# Autodesk Inventor assembly: MainDriveTestRig
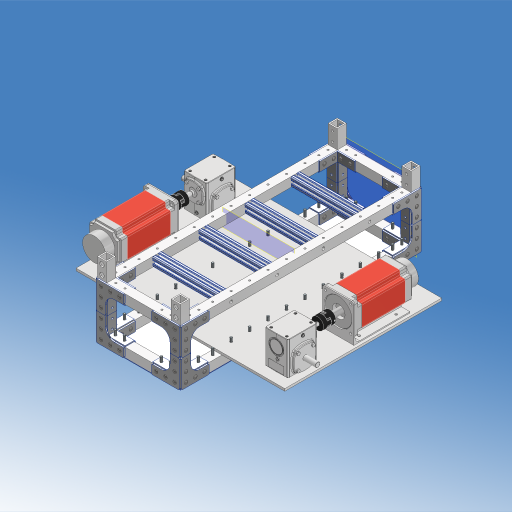
[picture p0: Inventor's stored thumbnail of the model, 512x512]
Saved by Autodesk Inventor 2024 (Build 280153000, 153)
## iProperties
Created: 2024-02-14
Part Number: MainDriveTestRig
Document SubType Name: Assembly
Designer: seene
Author: seene
## Documents named in this file (10)
- C:\Users\seene\OneDrive\SBRT\Robocup Rescue\Drive\TestRigs\MainDriveTestrig\MainDriveTestRig.iam
- C:\Users\seene\OneDrive\SBRT\Robocup Rescue\Chassis\Frame\Centerpiece\Centerpiece_Frame.iam
- Centerpiece_Frame.iam
- C:\Users\seene\OneDrive\SBRT\Robocup Rescue\Drive\v1\QCI-34HC-3_v2.ipt
- C:\Users\seene\OneDrive\SBRT\Robocup Rescue\Drive\v1\5887K171_Right-Angle Speed Reducer.ipt
- C:\Users\seene\OneDrive\SBRT\Robocup Rescue\Drive\v1\9939T12_Durometer 64D Spider for 1-5 16 OD Set Screw Vibrate-Damping Precision Flexible Shaft Coupling.ipt
- C:\Users\seene\OneDrive\SBRT\Robocup Rescue\Drive\v1\9939T102_Vibrate-Damping Precision Flexible Shaft Coupling.ipt
- C:\Users\seene\OneDrive\SBRT\Robocup Rescue\Drive\v1\9939T104_Vibrate-Damping Precision Flexible Shaft Coupling.ipt
- C:\Users\seene\OneDrive\SBRT\Robocup Rescue\Drive\TestRigs\MainDriveTestrig\MotorAttachementPlate.ipt
- C:\Users\seene\OneDrive\SBRT\Robocup Rescue\Drive\TestRigs\MainDriveTestrig\MotorStandoff.ipt
## Components (14 placed, 8 different names)
1. Centerpiece_Frame:1 [sub-assembly] — Mate:22, Mate:23, Mate:24
2. QCI-34HC-3_v2:2 — Rigid:1, Mate:21, Angle:1, Symmetry:2, Flush:30, Mate:30, Mate:31
3. 5887K171_Right-Angle Speed Reducer:1 — Mate:6, Mate:7, Flush:7, Mate:26, Flush:8
4. 9939T102_Vibrate-Damping Precision Flexible Shaft Coupling:1 — Mate:1, Mate:2, Mate:3, Mate:4, Mate:6, Mate:7
5. 9939T104_Vibrate-Damping Precision Flexible Shaft Coupling:1 — Mate:1, Mate:2, Mate:5, Rigid:1
6. 9939T12_Durometer 64D Spider for 1-5 16 OD Set Screw Vibrate-Damping Precision Flexible Shaft Coupling:2 — Mate:3, Mate:4, Mate:5
7. QCI-34HC-3_v2:3 — Mate:19, Mate:20, Symmetry:1, Mate:25, Flush:29, Mate:29
8. 5887K171_Right-Angle Speed Reducer:3 — Flush:3, Flush:6, Mate:27
9. 9939T102_Vibrate-Damping Precision Flexible Shaft Coupling:3
10. 9939T104_Vibrate-Damping Precision Flexible Shaft Coupling:3
11. 9939T12_Durometer 64D Spider for 1-5 16 OD Set Screw Vibrate-Damping Precision Flexible Shaft Coupling:3
12. MotorAttachementPlate:1 — Mate:22, Mate:23, Mate:24, Mate:25, Flush:6, Flush:7, Mate:26, Mate:27, Flush:8
13. MotorStandoff:1 — Flush:29, Mate:29
14. MotorStandoff:2 — Flush:30, Mate:30, Mate:31
## Relationships (39: Mate 26, Flush 8, WeldJoint 2, Symmetry 2, Angle 1)
- Mate:1: 9939T102_Vibrate-Damping Precision Flexible Shaft Coupling:1 ↔ 9939T104_Vibrate-Damping Precision Flexible Shaft Coupling:1
- Mate:2: 9939T102_Vibrate-Damping Precision Flexible Shaft Coupling:1 ↔ 9939T104_Vibrate-Damping Precision Flexible Shaft Coupling:1
- Mate:3: 9939T102_Vibrate-Damping Precision Flexible Shaft Coupling:1 ↔ 9939T12_Durometer 64D Spider for 1-5 16 OD Set Screw Vibrate-Damping Precision Flexible Shaft Coupling:2
- Mate:4: 9939T102_Vibrate-Damping Precision Flexible Shaft Coupling:1 ↔ 9939T12_Durometer 64D Spider for 1-5 16 OD Set Screw Vibrate-Damping Precision Flexible Shaft Coupling:2
- Mate:5: 9939T104_Vibrate-Damping Precision Flexible Shaft Coupling:1 ↔ 9939T12_Durometer 64D Spider for 1-5 16 OD Set Screw Vibrate-Damping Precision Flexible Shaft Coupling:2
- Rigid:1 [WeldJoint]: QCI-34HC-3_v2:2 ↔ 9939T104_Vibrate-Damping Precision Flexible Shaft Coupling:1
- Mate:6: 5887K171_Right-Angle Speed Reducer:1 ↔ 9939T102_Vibrate-Damping Precision Flexible Shaft Coupling:1
- Mate:7: 5887K171_Right-Angle Speed Reducer:1 ↔ 9939T102_Vibrate-Damping Precision Flexible Shaft Coupling:1
- [Mate]: 9939T102_Vibrate-Damping Precision Flexible Shaft Coupling:3 ↔ 9939T104_Vibrate-Damping Precision Flexible Shaft Coupling:3
- [Mate]: 9939T102_Vibrate-Damping Precision Flexible Shaft Coupling:3 ↔ 9939T104_Vibrate-Damping Precision Flexible Shaft Coupling:3
- [Mate]: 9939T102_Vibrate-Damping Precision Flexible Shaft Coupling:3 ↔ 9939T12_Durometer 64D Spider for 1-5 16 OD Set Screw Vibrate-Damping Precision Flexible Shaft Coupling:3
- [Mate]: 9939T102_Vibrate-Damping Precision Flexible Shaft Coupling:3 ↔ 9939T12_Durometer 64D Spider for 1-5 16 OD Set Screw Vibrate-Damping Precision Flexible Shaft Coupling:3
- [Mate]: 9939T104_Vibrate-Damping Precision Flexible Shaft Coupling:3 ↔ 9939T12_Durometer 64D Spider for 1-5 16 OD Set Screw Vibrate-Damping Precision Flexible Shaft Coupling:3
- [WeldJoint]: QCI-34HC-3_v2:3 ↔ 9939T104_Vibrate-Damping Precision Flexible Shaft Coupling:3
- [Mate]: 5887K171_Right-Angle Speed Reducer:3 ↔ 9939T102_Vibrate-Damping Precision Flexible Shaft Coupling:3
- [Mate]: 5887K171_Right-Angle Speed Reducer:3 ↔ 9939T102_Vibrate-Damping Precision Flexible Shaft Coupling:3
- Mate:19: QCI-34HC-3_v2:3
- Mate:20: QCI-34HC-3_v2:3
- Symmetry:1: QCI-34HC-3_v2:3
- Flush:3 (-33.274 mm): 5887K171_Right-Angle Speed Reducer:3
- Flush:4
- Mate:21: QCI-34HC-3_v2:2
- Angle:1 (0 deg): QCI-34HC-3_v2:2
- Symmetry:2: QCI-34HC-3_v2:2
- Flush:5
- Mate:22: Centerpiece_Frame:1 ↔ MotorAttachementPlate:1
- Mate:23: Centerpiece_Frame:1 ↔ MotorAttachementPlate:1
- Mate:24: Centerpiece_Frame:1 ↔ MotorAttachementPlate:1
- Mate:25: QCI-34HC-3_v2:3 ↔ MotorAttachementPlate:1
- Flush:6 (12.7 mm): 5887K171_Right-Angle Speed Reducer:3 ↔ MotorAttachementPlate:1
- Flush:7 (12.7 mm): 5887K171_Right-Angle Speed Reducer:1 ↔ MotorAttachementPlate:1
- Mate:26: 5887K171_Right-Angle Speed Reducer:1 ↔ MotorAttachementPlate:1
- Mate:27: 5887K171_Right-Angle Speed Reducer:3 ↔ MotorAttachementPlate:1
- Flush:8: 5887K171_Right-Angle Speed Reducer:1 ↔ MotorAttachementPlate:1
- Flush:29: QCI-34HC-3_v2:3 ↔ MotorStandoff:1
- Mate:29: QCI-34HC-3_v2:3 ↔ MotorStandoff:1
- Flush:30: QCI-34HC-3_v2:2 ↔ MotorStandoff:2
- Mate:30: QCI-34HC-3_v2:2 ↔ MotorStandoff:2
- Mate:31: QCI-34HC-3_v2:2 ↔ MotorStandoff:2
## Named parameters: d11_d3 = 0 mm, d12_d4 = 0 mm, d13_d5 = 0 mm, d14_d6 = 0 mm, d15_d7 = 0 mm, d16_d8 = 0 mm, d17_d9 = 0 mm, d18_d10 = 0 mm
